# Autodesk Inventor assembly: ParticleLauncherwCollector
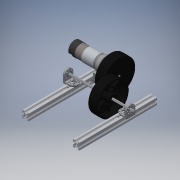
[picture p0: Inventor's stored thumbnail of the model, 180x180]
Saved by Autodesk Inventor 2016 (Build 200138000, 138)
## iProperties
Created: 2016-10-12
Part Number: ParticleLauncherwCollector
Document SubType Name: Assembly
Designer: Delta
Author: Delta
## Documents named in this file (9)
- C:\Robotics\CAD\2016-17_CAD\ParticleLauncherwCollector.iam
- C:\Robotics\CAD\COTSParts\Actobotics\555 parts\555116.ipt
- C:\Robotics\CAD\COTSParts\Actobotics\am-3102NeveRest20 (1).ipt
- C:\Robotics\CAD\COTSParts\Actobotics\634 parts\634088.ipt
- C:\Robotics\CAD\COTSParts\Wheels\4in Wheel Intergreated Hub 8mm Rev2.ipt
- C:\Robotics\CAD\COTSParts\Bosch Extrusion\Bosch 20x20 9 in.ipt
- C:\Robotics\CAD\COTSParts\Bearings - AndyMark\Bearing 250 ID 500 OD flanged.ipt
- C:\Robotics\CAD\COTSParts\Actobotics\545 parts\545400.ipt
- C:\Robotics\CAD\COTSParts\Bosch Extrusion\6mm block nut M4.ipt
## Components (18 placed, 8 different names)
1. 555116:1 — Insert:15, Flush:5, Mate:1, Flush:6
2. am-3102NeveRest20 (1):1 — Insert:15, Insert:18
3. 634088:1 — Insert:17, Insert:30, Insert:31
4. 4in Wheel Intergreated Hub 8mm Rev2:1 — Insert:17
5. 4in Wheel Intergreated Hub 8mm Rev2:2 — Insert:18
6. Bosch 20x20 9 in:1 — Mate:3, Mate:4, Mate:5, Mate:7, Mate:8, Mate:9, Mate:10, Flush:7, Flush:8, Flush:9
7. Bosch 20x20 9 in:2 — Mate:11, Mate:12, Mate:13, Mate:14, Flush:8, Flush:9
8. Bearing 250 ID 500 OD flanged:2 — Mate:15, Insert:29, Insert:30
9. Bearing 250 ID 500 OD flanged:3 — Insert:31, Insert:32
10. 545400:1 — Insert:23, Insert:24, Insert:32
11. 545400:2 — Insert:27, Insert:28, Mate:15, Insert:29
12. 545400:8 — Flush:5, Mate:1, Insert:19, Insert:20, Flush:6
13. 6mm block nut M4:1 — Mate:3, Mate:4, Insert:19, Flush:7
14. 6mm block nut M4:2 — Insert:20, Mate:5
15. 6mm block nut M4:4 — Mate:7, Mate:8, Insert:23
16. 6mm block nut M4:5 — Mate:9, Mate:10, Insert:24
17. 6mm block nut M4:6 — Mate:13, Mate:14, Insert:28
18. 6mm block nut M4:7 — Mate:11, Mate:12, Insert:27
## Relationships (31: Insert 13, Mate 13, Flush 5)
- Insert:15 (-9.525 mm): 555116:1 ↔ am-3102NeveRest20 (1):1
- Insert:17 (63.5 mm): 634088:1 ↔ 4in Wheel Intergreated Hub 8mm Rev2:1
- Insert:18: am-3102NeveRest20 (1):1 ↔ 4in Wheel Intergreated Hub 8mm Rev2:2
- Flush:5 (4.0386 mm): 555116:1 ↔ 545400:8
- Mate:1: 555116:1 ↔ 545400:8
- Mate:3: Bosch 20x20 9 in:1 ↔ 6mm block nut M4:1
- Mate:4: Bosch 20x20 9 in:1 ↔ 6mm block nut M4:1
- Insert:19: 545400:8 ↔ 6mm block nut M4:1
- Insert:20: 545400:8 ↔ 6mm block nut M4:2
- Mate:5: Bosch 20x20 9 in:1 ↔ 6mm block nut M4:2
- Flush:6 (14.2748 mm): 555116:1 ↔ 545400:8
- Mate:7: Bosch 20x20 9 in:1 ↔ 6mm block nut M4:4
- Mate:8: Bosch 20x20 9 in:1 ↔ 6mm block nut M4:4
- Insert:23: 545400:1 ↔ 6mm block nut M4:4
- Mate:9: Bosch 20x20 9 in:1 ↔ 6mm block nut M4:5
- Mate:10: Bosch 20x20 9 in:1 ↔ 6mm block nut M4:5
- Insert:24: 545400:1 ↔ 6mm block nut M4:5
- Mate:11: Bosch 20x20 9 in:2 ↔ 6mm block nut M4:7
- Mate:12: Bosch 20x20 9 in:2 ↔ 6mm block nut M4:7
- Insert:27: 545400:2 ↔ 6mm block nut M4:7
- Mate:13: Bosch 20x20 9 in:2 ↔ 6mm block nut M4:6
- Mate:14: Bosch 20x20 9 in:2 ↔ 6mm block nut M4:6
- Insert:28: 545400:2 ↔ 6mm block nut M4:6
- Flush:7 (-10.668 mm): Bosch 20x20 9 in:1 ↔ 6mm block nut M4:1
- Flush:8: Bosch 20x20 9 in:1 ↔ Bosch 20x20 9 in:2
- Mate:15: Bearing 250 ID 500 OD flanged:2 ↔ 545400:2
- Insert:29: Bearing 250 ID 500 OD flanged:2 ↔ 545400:2
- Insert:30 (12.225 mm): 634088:1 ↔ Bearing 250 ID 500 OD flanged:2
- Insert:31 (13.241 mm): 634088:1 ↔ Bearing 250 ID 500 OD flanged:3
- Insert:32: Bearing 250 ID 500 OD flanged:3 ↔ 545400:1
- Flush:9: Bosch 20x20 9 in:1 ↔ Bosch 20x20 9 in:2
